# Autodesk Inventor assembly: fan-assembly
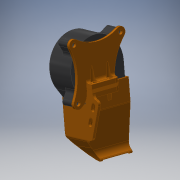
[picture p0: Inventor's stored thumbnail of the model, 180x180]
Saved by Autodesk Inventor 2018 (Build 220112000, 112)
## iProperties
Created: 2020-01-13
Part Number: fan-assembly
Document SubType Name: Assembly
Designer: Vinnie Caprarola
Author: Vinnie Caprarola
## Documents named in this file (4)
- Z:\Z\custom-parts\fan\fan-assembly.iam
- Z:\Z\custom-parts\fan\4020-blower-fan.ipt
- Z:\Z\custom-parts\fan\40mm_blower_fan_shroud.ipt
- Z:\Z\custom-parts\fan\fan-mount-plate.ipt
## Components (3 placed, 3 different names)
1. 4020-blower-fan:1 — Mate:1, Mate:2, Mate:3, Flush:1, Flush:2, Flush:3
2. 40mm_blower_fan_shroud:1 — Mate:1, Mate:2, Mate:3, Flush:4
3. fan-mount-plate:1 — Flush:1, Flush:2, Flush:3, Flush:4
## Relationships (7: Flush 4, Mate 3)
- Mate:1: 4020-blower-fan:1 ↔ 40mm_blower_fan_shroud:1
- Mate:2: 4020-blower-fan:1 ↔ 40mm_blower_fan_shroud:1
- Mate:3: 4020-blower-fan:1 ↔ 40mm_blower_fan_shroud:1
- Flush:1: 4020-blower-fan:1 ↔ fan-mount-plate:1
- Flush:2: 4020-blower-fan:1 ↔ fan-mount-plate:1
- Flush:3: 4020-blower-fan:1 ↔ fan-mount-plate:1
- Flush:4: 40mm_blower_fan_shroud:1 ↔ fan-mount-plate:1
